# Autodesk Inventor assembly: ElvatorBottom
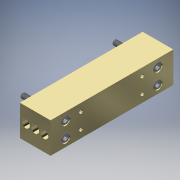
[picture p0: Inventor's stored thumbnail of the model, 180x180]
Saved by Autodesk Inventor 2019 (Build 230136000, 136)
## iProperties
Created: 2019-09-28
Part Number: ElvatorBottom
Document SubType Name: Assembly
Designer: james
Author: james
## Documents named in this file (3)
- F:\JimsDesign\Jims2020FTC\ElvatorBottom.iam
- F:\JimsDesign\Library\McMaster\SocketScrews\91251A201_BLACK-OXIDE ALLOY STEEL SOCKET HEAD SCREW.ipt
- F:\JimsDesign\Jims2020FTC\BottomOfBackElevatorFrame.ipt
## Components (5 placed, 2 different names)
1. BottomOfBackElevatorFrame:1 — Mate:1, Mate:2, Mate:3, Mate:4, Mate:5, Mate:6, Mate:7, Mate:8
2. 91251A201_BLACK-OXIDE ALLOY STEEL SOCKET HEAD SCREW:1 — Mate:3, Mate:4
3. 91251A201_BLACK-OXIDE ALLOY STEEL SOCKET HEAD SCREW:2 — Mate:1, Mate:2
4. 91251A201_BLACK-OXIDE ALLOY STEEL SOCKET HEAD SCREW:3 — Mate:6, Mate:7
5. 91251A201_BLACK-OXIDE ALLOY STEEL SOCKET HEAD SCREW:4 — Mate:5, Mate:8
## Relationships (8: Mate 8)
- Mate:1: BottomOfBackElevatorFrame:1 ↔ 91251A201_BLACK-OXIDE ALLOY STEEL SOCKET HEAD SCREW:2
- Mate:2: BottomOfBackElevatorFrame:1 ↔ 91251A201_BLACK-OXIDE ALLOY STEEL SOCKET HEAD SCREW:2
- Mate:3: BottomOfBackElevatorFrame:1 ↔ 91251A201_BLACK-OXIDE ALLOY STEEL SOCKET HEAD SCREW:1
- Mate:4: BottomOfBackElevatorFrame:1 ↔ 91251A201_BLACK-OXIDE ALLOY STEEL SOCKET HEAD SCREW:1
- Mate:5: BottomOfBackElevatorFrame:1 ↔ 91251A201_BLACK-OXIDE ALLOY STEEL SOCKET HEAD SCREW:4
- Mate:6: BottomOfBackElevatorFrame:1 ↔ 91251A201_BLACK-OXIDE ALLOY STEEL SOCKET HEAD SCREW:3
- Mate:7: BottomOfBackElevatorFrame:1 ↔ 91251A201_BLACK-OXIDE ALLOY STEEL SOCKET HEAD SCREW:3
- Mate:8: BottomOfBackElevatorFrame:1 ↔ 91251A201_BLACK-OXIDE ALLOY STEEL SOCKET HEAD SCREW:4
